# Autodesk Inventor assembly: MaquinaDeCorte
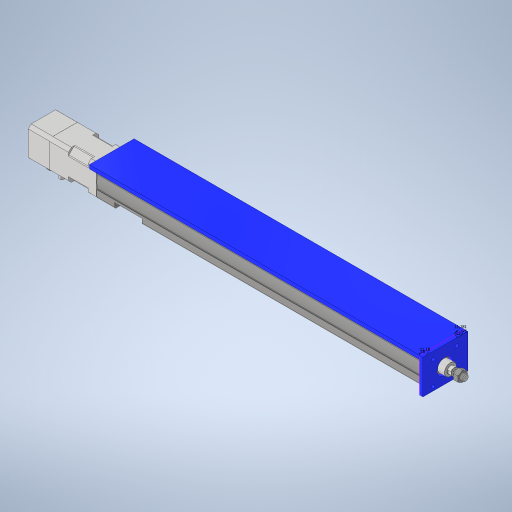
[picture p0: Inventor's stored thumbnail of the model, 512x512]
Saved by Autodesk Inventor 2023 (Build 270158000, 158)
## iProperties
Created: 2023-04-07
Part Number: MaquinaDeCorte
Document SubType Name: Assembly
Designer: Lenovo
Author: Lenovo
## Documents named in this file (3)
- D:\Esdek\Gemelo Digital\Corte de Tubos\MaquinaDeCorte.iam
- D:\Esdek\Gemelo Digital\Corte de Tubos\CADimportados\PistónElectromecánico\1470706 EPCO-25-300-3P-ST-E---(0).iam
- D:\Esdek\Gemelo Digital\Corte de Tubos\SoporteElectromecánico.ipt
## Components (2 placed, 2 different names)
1. 1470706 EPCO-25-300-3P-ST-E---(0):1 [sub-assembly] — Mate:1, Mate:2, Mate:3
2. SoporteElectromecánico:1 — Mate:1, Mate:2, Mate:3
## Relationships (3: Mate 3)
- Mate:1: 1470706 EPCO-25-300-3P-ST-E---(0):1 ↔ SoporteElectromecánico:1
- Mate:2: 1470706 EPCO-25-300-3P-ST-E---(0):1 ↔ SoporteElectromecánico:1
- Mate:3: 1470706 EPCO-25-300-3P-ST-E---(0):1 ↔ SoporteElectromecánico:1
